# Autodesk Inventor assembly: CableBraider
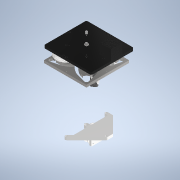
[picture p0: Inventor's stored thumbnail of the model, 180x180]
Saved by Autodesk Inventor 2022 (Build 260153000, 153)
## iProperties
Created: 2020-07-21
Part Number: CableBraider
Document SubType Name: Assembly
Designer: elmar
Author: elmar
## Documents named in this file (12)
- C:\repo\FourWireBraidingMachine\MetalCableBraider\CableBraider.iam
- C:\repo\FourWireBraidingMachine\MetalCableBraider\BasePlate.ipt
- C:\repo\FourWireBraidingMachine\MetalCableBraider\WinderAssembly.iam
- C:\repo\FourWireBraidingMachine\MetalCableBraider\Carriage.iam
- C:\repo\FourWireBraidingMachine\MetalCableBraider\NEMA17.ipt
- C:\repo\FourWireBraidingMachine\MetalCableBraider\ElectronicsPlate.ipt
- C:\repo\FourWireBraidingMachine\MetalCableBraider\DriveGearNEMA17.ipt
- C:\repo\FourWireBraidingMachine\MetalCableBraider\TwoPartHornGear.ipt
- C:\repo\FourWireBraidingMachine\MetalCableBraider\GuidePlate.ipt
- C:\repo\FourWireBraidingMachine\MetalCableBraider\HornGearShaft.ipt
- C:\Users\Eric\OneDrive\Documents\Inventor\Content Center Files\R2022\en-US\DIN 934\DIN 934 - M8 x 1.25.ipt
- C:\Users\Eric\OneDrive\Documents\Inventor\Content Center Files\R2022\en-US\DIN 934\DIN 934 - M7 x 1.ipt
## Components (14 placed, 11 different names)
1. BasePlate:1 — Mate:1, Mate:2, Mate:3, Mate:10, Mate:13, Angle:5, Mate:14, Insert:1, Insert:2, Mate:16, Insert:4, Insert:6, Insert:7
2. TwoPartHornGear:1 — Angle:3, Flush:3, Insert:2, Flush:4
3. TwoPartHornGear:2 — Angle:3, Mate:16, Flush:4
4. WinderAssembly:1 [sub-assembly]
5. Carriage:1 [sub-assembly] — Mate:15
6. NEMA17:1 — Mate:10, Mate:12, Angle:4, Insert:1
7. ElectronicsPlate:1
8. DriveGearNEMA17:1 — Mate:12, Flush:3, Angle:4
9. GuidePlate:1 — Mate:13, Angle:5, Mate:14, Mate:15, Insert:3, Angle:6, Angle:7, Insert:5
10. HornGearShaft:1 — Insert:3, Angle:6
11. HornGearShaft:2 — Angle:7, Insert:4
12. DIN 934 - replaced by DIN EN 24032/28673/28674 M8:1 — Insert:5
13. DIN 934 - replaced by DIN EN 24032/28673/28674 M7:1 — Insert:6
14. DIN 934 - replaced by DIN EN 24032/28673/28674 M7:5 — Insert:7
## Relationships (23: Mate 9, Insert 7, Angle 5, Flush 2)
- Mate:1: BasePlate:1
- Mate:2: BasePlate:1
- Mate:3: BasePlate:1
- Angle:3 (0 deg): TwoPartHornGear:1 ↔ TwoPartHornGear:2
- Mate:10: BasePlate:1 ↔ NEMA17:1
- Mate:12: NEMA17:1 ↔ DriveGearNEMA17:1
- Flush:3: TwoPartHornGear:1 ↔ DriveGearNEMA17:1
- Angle:4 (180 deg): NEMA17:1 ↔ DriveGearNEMA17:1
- Mate:13: BasePlate:1 ↔ GuidePlate:1
- Angle:5 (0 deg): BasePlate:1 ↔ GuidePlate:1
- Mate:14 (40 mm): BasePlate:1 ↔ GuidePlate:1
- Mate:15: Carriage:1 ↔ GuidePlate:1
- Insert:1: BasePlate:1 ↔ NEMA17:1
- Insert:2 (1.6 mm): BasePlate:1 ↔ TwoPartHornGear:1
- Mate:16: BasePlate:1 ↔ TwoPartHornGear:2
- Flush:4: TwoPartHornGear:1 ↔ TwoPartHornGear:2
- Insert:3: GuidePlate:1 ↔ HornGearShaft:1
- Angle:6 (180 deg): GuidePlate:1 ↔ HornGearShaft:1
- Angle:7 (180 deg): GuidePlate:1 ↔ HornGearShaft:2
- Insert:4: BasePlate:1 ↔ HornGearShaft:2
- Insert:5: GuidePlate:1 ↔ DIN 934 - replaced by DIN EN 24032/28673/28674 M8:1
- Insert:6: BasePlate:1 ↔ DIN 934 - replaced by DIN EN 24032/28673/28674 M7:1
- Insert:7: BasePlate:1 ↔ DIN 934 - replaced by DIN EN 24032/28673/28674 M7:5
